# Autodesk Inventor assembly: 右脚ユニット3
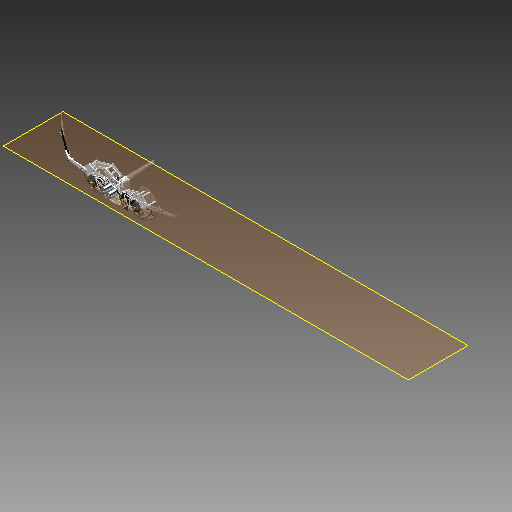
[picture p0: Inventor's stored thumbnail of the model, 512x512]
Saved by Autodesk Inventor 2020 (Build 240168000, 168)
## iProperties
Created: 2019-09-04
Part Number: 右脚ユニット3
Document SubType Name: Assembly
Designer: 雪村
Mass: 941.287 g
Surface Area: 4355.6 cm^2
Volume: 381.334 cm^3
Density: 2.46841 g/cm^3
Author: 雪村
## Documents named in this file (6)
- C:\Users\white\Documents\SRDC\SRDC\Inventor_2017\2018年機体\2020年4年機体\右脚ユニット3.iam
- C:\Users\white\Documents\SRDC\SRDC\Inventor_2017\2018年機体\2020年4年機体\右脚中間ユニット2.iam
- C:\Users\white\Documents\SRDC\SRDC\Inventor_2017\2018年機体\2020年4年機体\右後脚ユニット5.iam
- C:\Users\white\Documents\SRDC\SRDC\Inventor_2017\2018年機体\2020年4年機体\右前脚ユニット5.iam
- C:\Users\white\Documents\SRDC\SRDC\Inventor_2017\2018年機体\2020年4年機体\平行サスシャフト4.iam
- C:\Users\white\Documents\SRDC\SRDC\Inventor_2017\2018年機体\パーツ\タミヤダンパー.iam
## Components (6 placed, 5 different names)
1. 右脚中間ユニット2:1 [sub-assembly] — フラッシュ:1, 挿入:1, 挿入:2, メイト:1, 挿入:7, メイト:4
2. 右後脚ユニット5:1 [sub-assembly] — 挿入:1, メイト:3
3. 右前脚ユニット5:1 [sub-assembly] — 挿入:2, 挿入:5
4. 平行サスシャフト4:1 [sub-assembly] — メイト:1, 挿入:5, 挿入:6
5. タミヤダンパー:1 [sub-assembly] — 挿入:6, メイト:4
6. タミヤダンパー:2 [sub-assembly] — 挿入:7, メイト:3
## Relationships (10: Insert 5, Mate 3, Flush 2)
- フラッシュ:1 [Flush] (-130 mm): 右脚中間ユニット2:1
- 挿入:1 [Insert]: 右脚中間ユニット2:1 ↔ 右後脚ユニット5:1
- 挿入:2 [Insert]: 右脚中間ユニット2:1 ↔ 右前脚ユニット5:1
- メイト:1 [Mate]: 右脚中間ユニット2:1 ↔ 平行サスシャフト4:1
- 挿入:5 [Insert]: 右前脚ユニット5:1 ↔ 平行サスシャフト4:1
- 挿入:6 [Insert] (10 mm): 平行サスシャフト4:1 ↔ タミヤダンパー:1
- 挿入:7 [Insert] (4 mm): 右脚中間ユニット2:1 ↔ タミヤダンパー:2
- メイト:3 [Mate]: 右後脚ユニット5:1 ↔ タミヤダンパー:2
- メイト:4 [Mate]: 右脚中間ユニット2:1 ↔ タミヤダンパー:1
- フラッシュ:2 [Flush] (70 mm)
